# Autodesk Inventor assembly: Impresora 3D
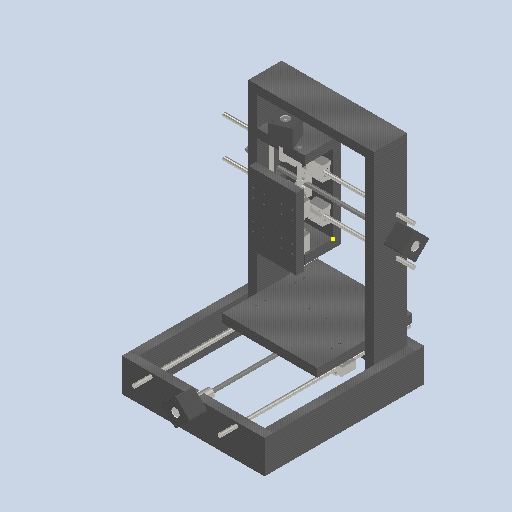
[picture p0: Inventor's stored thumbnail of the model, 512x512]
Saved by Autodesk Inventor 2022.2 (Build 262287000, 287)
## iProperties
Created: 2021-11-08
Part Number: Impresora 3D
Document SubType Name: Assembly
Designer: Samuel Gómez
Author: Samuel Gómez
## Documents named in this file (16)
- E:\Samuel Gómez\Documentos\ITM\Cuarto Semestre\Dibujo\Final\Original\Trabajo Final Impresora 3D\Impresora 3D.iam
- E:\Samuel Gómez\Documentos\ITM\Cuarto Semestre\Dibujo\Final\Original\Trabajo Final Impresora 3D\Placa1.ipt
- E:\Samuel Gómez\Documentos\ITM\Cuarto Semestre\Dibujo\Final\Original\Trabajo Final Impresora 3D\Placa2.ipt
- E:\Samuel Gómez\Documentos\ITM\Cuarto Semestre\Dibujo\Final\Original\Trabajo Final Impresora 3D\Placa1 Tracera.ipt
- E:\Samuel Gómez\Documentos\ITM\Cuarto Semestre\Dibujo\Final\Original\Trabajo Final Impresora 3D\Placa4 Torre.ipt
- E:\Samuel Gómez\Documentos\ITM\Cuarto Semestre\Dibujo\Final\Original\Trabajo Final Impresora 3D\Placa4 Torre Tracera.ipt
- E:\Samuel Gómez\Documentos\ITM\Cuarto Semestre\Dibujo\Final\Original\Trabajo Final Impresora 3D\Varrilla.ipt
- E:\Samuel Gómez\Documentos\ITM\Cuarto Semestre\Dibujo\Final\Original\Trabajo Final Impresora 3D\REFUERZO.ipt
- E:\Samuel Gómez\Documentos\ITM\Cuarto Semestre\Dibujo\Final\Original\Trabajo Final Impresora 3D\Balero lineal.ipt
- E:\Samuel Gómez\Documentos\ITM\Cuarto Semestre\Dibujo\Final\Original\Trabajo Final Impresora 3D\MOTOR.ipt
- E:\Samuel Gómez\Documentos\ITM\Cuarto Semestre\Dibujo\Final\Original\Trabajo Final Impresora 3D\ACOPLE FLEXIBLE.ipt
- E:\Samuel Gómez\Documentos\ITM\Cuarto Semestre\Dibujo\Final\Original\Trabajo Final Impresora 3D\Placa3 Cama.ipt
- E:\Samuel Gómez\Documentos\ITM\Cuarto Semestre\Dibujo\Final\Original\Trabajo Final Impresora 3D\CAMISA.ipt
- E:\Samuel Gómez\Documentos\ITM\Cuarto Semestre\Dibujo\Final\Original\Trabajo Final Impresora 3D\Extrusor.iam
- E:\Samuel Gómez\Documentos\ITM\Cuarto Semestre\Dibujo\Final\Original\Trabajo Final Impresora 3D\Placa5 Base Extrusor.ipt
- E:\Samuel Gómez\Documentos\ITM\Cuarto Semestre\Dibujo\Final\Original\Trabajo Final Impresora 3D\TORNILLO.ipt
## Components (36 placed, 15 different names)
1. Placa1:1 — Coincidencia:1, Nivelación:1, Nivelación:2, Nivelación:3, Nivelación:4, Coincidencia:2, Coincidencia:8, Coincidencia:9, Nivelación:9, Nivelación:10, Coincidencia:21, Coincidencia:22, Coincidencia:23
2. Placa2:1 — Coincidencia:1, Nivelación:1, Nivelación:2, Coincidencia:3, Coincidencia:4, Ángulo:3, Ángulo:4
3. Placa2:2 — Nivelación:3, Nivelación:4, Coincidencia:2, Nivelación:5, Nivelación:6, Coincidencia:6, Nivelación:8, Ángulo:1, Ángulo:2
4. Placa1 Tracera:1 — Coincidencia:3, Nivelación:5, Nivelación:6, Coincidencia:5, Nivelación:7, Coincidencia:7, Coincidencia:60
5. Placa4 Torre:1 — Coincidencia:4, Coincidencia:5, Nivelación:7, Nivelación:11, Nivelación:14, Coincidencia:24, Coincidencia:25, Coincidencia:26, Ángulo:11, Ángulo:12
6. Placa4 Torre Tracera:1 — Coincidencia:6, Coincidencia:7, Nivelación:8, Coincidencia:10, Coincidencia:11, Coincidencia:12, Nivelación:13, Ángulo:9, Ángulo:10, Coincidencia:61
7. Varrilla:1 — Coincidencia:8, Nivelación:10, Coincidencia:13, Coincidencia:14
8. Varrilla:2 — Coincidencia:9, Nivelación:9, Coincidencia:15, Coincidencia:16
9. Varrilla:3 — Coincidencia:10, Nivelación:11, Nivelación:12, Coincidencia:17, Coincidencia:19
10. Varrilla:4 — Coincidencia:11, Nivelación:12, Coincidencia:18, Coincidencia:20
11. Refuerzo:1 — Coincidencia:12, Nivelación:13, Nivelación:14, Ángulo:5, Ángulo:6, Ángulo:7, Ángulo:8
12. Balero lineal:1 — Coincidencia:13, Ángulo:1, Nivelación:16, Coincidencia:31
13. Balero lineal:2 — Coincidencia:14, Ángulo:2, Nivelación:15, Coincidencia:30, Coincidencia:60
14. Balero lineal:3 — Coincidencia:15, Ángulo:3, Nivelación:15
15. Balero lineal:4 — Coincidencia:16, Ángulo:4, Nivelación:16, Coincidencia:29
16. Balero lineal:5 — Coincidencia:18, Ángulo:6, Nivelación:17, Coincidencia:35, Coincidencia:36, Coincidencia:37
17. Balero lineal:6 — Coincidencia:17, Ángulo:5, Nivelación:17, Coincidencia:38
18. Balero lineal:7 — Coincidencia:20, Ángulo:7, Nivelación:18
19. Balero lineal:8 — Coincidencia:19, Ángulo:8, Nivelación:18, Coincidencia:39
20. Motor:1 — Coincidencia:21, Coincidencia:22, Coincidencia:23, Coincidencia:27, Nivelación:19
21. Motor:2 — Coincidencia:24, Coincidencia:25, Coincidencia:26, Coincidencia:28, Nivelación:20
22. Acople Flexible:1 — Coincidencia:27, Nivelación:19, Coincidencia:55, Coincidencia:56
23. Acople Flexible:2 — Coincidencia:28, Nivelación:20, Coincidencia:53, Coincidencia:54
24. Placa3 Cama:1 — Coincidencia:29, Coincidencia:30, Coincidencia:31, Coincidencia:32, Coincidencia:33, Coincidencia:34
25. Camisa:1 — Coincidencia:32, Coincidencia:33, Coincidencia:34
26. Extrusor:1 [sub-assembly] — Coincidencia:35, Coincidencia:36, Coincidencia:37, Coincidencia:38, Coincidencia:39, Coincidencia:40, Coincidencia:41, Coincidencia:42, Coincidencia:44, Coincidencia:45, Coincidencia:46, Coincidencia:47, Coincidencia:52, Coincidencia:57, Coincidencia:58, Coincidencia:59, Coincidencia:61
27. Motor:3 — Coincidencia:40, Coincidencia:41, Coincidencia:42, Coincidencia:43, Nivelación:21
28. Acople Flexible:3 — Coincidencia:43, Nivelación:21
29. Balero lineal:9 — Coincidencia:46, Ángulo:9, Nivelación:22
30. Balero lineal:10 — Coincidencia:45, Ángulo:12, Nivelación:23, Coincidencia:51, Coincidencia:52
31. Balero lineal:11 — Coincidencia:44, Ángulo:11, Nivelación:22, Coincidencia:48, Coincidencia:49, Coincidencia:50
32. Balero lineal:12 — Coincidencia:47, Ángulo:10, Nivelación:23
33. Placa5 Base Extrusor:1 — Coincidencia:48, Coincidencia:49, Coincidencia:50, Coincidencia:51
34. Tornillo:1 — Coincidencia:53, Coincidencia:54
35. Tornillo:2 — Coincidencia:55, Coincidencia:56
36. Camisa:2 — Coincidencia:57, Coincidencia:58, Coincidencia:59
## Relationships (96: Mate 61, Flush 23, Angle 12)
- Coincidencia:1 [Mate]: Placa1:1 ↔ Placa2:1
- Nivelación:1 [Flush]: Placa1:1 ↔ Placa2:1
- Nivelación:2 [Flush]: Placa1:1 ↔ Placa2:1
- Nivelación:3 [Flush]: Placa1:1 ↔ Placa2:2
- Nivelación:4 [Flush]: Placa1:1 ↔ Placa2:2
- Coincidencia:2 [Mate]: Placa1:1 ↔ Placa2:2
- Coincidencia:3 [Mate]: Placa2:1 ↔ Placa1 Tracera:1
- Nivelación:5 [Flush]: Placa2:2 ↔ Placa1 Tracera:1
- Nivelación:6 [Flush]: Placa2:2 ↔ Placa1 Tracera:1
- Coincidencia:4 [Mate]: Placa2:1 ↔ Placa4 Torre:1
- Coincidencia:5 [Mate]: Placa1 Tracera:1 ↔ Placa4 Torre:1
- Nivelación:7 [Flush]: Placa1 Tracera:1 ↔ Placa4 Torre:1
- Coincidencia:6 [Mate]: Placa2:2 ↔ Placa4 Torre Tracera:1
- Coincidencia:7 [Mate]: Placa1 Tracera:1 ↔ Placa4 Torre Tracera:1
- Nivelación:8 [Flush]: Placa2:2 ↔ Placa4 Torre Tracera:1
- Coincidencia:8 [Mate]: Placa1:1 ↔ Varrilla:1
- Coincidencia:9 [Mate]: Placa1:1 ↔ Varrilla:2
- Nivelación:9 [Flush] (-35 mm): Placa1:1 ↔ Varrilla:2
- Nivelación:10 [Flush] (-35 mm): Placa1:1 ↔ Varrilla:1
- Coincidencia:10 [Mate]: Placa4 Torre Tracera:1 ↔ Varrilla:3
- Nivelación:11 [Flush] (35 mm): Placa4 Torre:1 ↔ Varrilla:3
- Coincidencia:11 [Mate]: Placa4 Torre Tracera:1 ↔ Varrilla:4
- Nivelación:12 [Flush]: Varrilla:3 ↔ Varrilla:4
- Coincidencia:12 [Mate]: Placa4 Torre Tracera:1 ↔ Refuerzo:1
- Nivelación:13 [Flush]: Placa4 Torre Tracera:1 ↔ Refuerzo:1
- Nivelación:14 [Flush]: Placa4 Torre:1 ↔ Refuerzo:1
- Coincidencia:13 [Mate]: Varrilla:1 ↔ Balero lineal:1
- Coincidencia:14 [Mate]: Varrilla:1 ↔ Balero lineal:2
- Ángulo:1 [Angle] (0 deg): Placa2:2 ↔ Balero lineal:1
- Ángulo:2 [Angle] (0 deg): Placa2:2 ↔ Balero lineal:2
- Coincidencia:15 [Mate]: Varrilla:2 ↔ Balero lineal:3
- Coincidencia:16 [Mate]: Varrilla:2 ↔ Balero lineal:4
- Ángulo:3 [Angle] (0 deg): Placa2:1 ↔ Balero lineal:3
- Ángulo:4 [Angle] (0 deg): Placa2:1 ↔ Balero lineal:4
- Nivelación:15 [Flush]: Balero lineal:2 ↔ Balero lineal:3
- Nivelación:16 [Flush]: Balero lineal:1 ↔ Balero lineal:4
- Coincidencia:17 [Mate]: Varrilla:3 ↔ Balero lineal:6
- Coincidencia:18 [Mate]: Varrilla:4 ↔ Balero lineal:5
- Ángulo:5 [Angle] (0 deg): Refuerzo:1 ↔ Balero lineal:6
- Ángulo:6 [Angle] (0 deg): Refuerzo:1 ↔ Balero lineal:5
- Nivelación:17 [Flush]: Balero lineal:5 ↔ Balero lineal:6
- Coincidencia:19 [Mate]: Varrilla:3 ↔ Balero lineal:8
- Coincidencia:20 [Mate]: Varrilla:4 ↔ Balero lineal:7
- Ángulo:7 [Angle] (0 deg): Refuerzo:1 ↔ Balero lineal:7
- Ángulo:8 [Angle] (0 deg): Refuerzo:1 ↔ Balero lineal:8
- Nivelación:18 [Flush]: Balero lineal:7 ↔ Balero lineal:8
- Coincidencia:21 [Mate]: Placa1:1 ↔ Motor:1
- Coincidencia:22 [Mate]: Placa1:1 ↔ Motor:1
- Coincidencia:23 [Mate]: Placa1:1 ↔ Motor:1
- Coincidencia:24 [Mate]: Placa4 Torre:1 ↔ Motor:2
- Coincidencia:25 [Mate]: Placa4 Torre:1 ↔ Motor:2
- Coincidencia:26 [Mate]: Placa4 Torre:1 ↔ Motor:2
- Coincidencia:27 [Mate]: Motor:1 ↔ Acople Flexible:1
- Nivelación:19 [Flush]: Motor:1 ↔ Acople Flexible:1
- Coincidencia:28 [Mate]: Motor:2 ↔ Acople Flexible:2
- Nivelación:20 [Flush]: Motor:2 ↔ Acople Flexible:2
- Coincidencia:29 [Mate]: Balero lineal:4 ↔ Placa3 Cama:1
- Coincidencia:30 [Mate]: Balero lineal:2 ↔ Placa3 Cama:1
- Coincidencia:31 [Mate]: Balero lineal:1 ↔ Placa3 Cama:1
- Coincidencia:32 [Mate]: Placa3 Cama:1 ↔ Camisa:1
- Coincidencia:33 [Mate]: Placa3 Cama:1 ↔ Camisa:1
- Coincidencia:34 [Mate]: Placa3 Cama:1 ↔ Camisa:1
- Coincidencia:35 [Mate]: Balero lineal:5 ↔ Extrusor:1
- Coincidencia:36 [Mate]: Balero lineal:5 ↔ Extrusor:1
- Coincidencia:37 [Mate]: Balero lineal:5 ↔ Extrusor:1
- Coincidencia:38 [Mate]: Balero lineal:6 ↔ Extrusor:1
- Coincidencia:39 [Mate]: Balero lineal:8 ↔ Extrusor:1
- Coincidencia:40 [Mate]: Extrusor:1 ↔ Motor:3
- Coincidencia:41 [Mate]: Extrusor:1 ↔ Motor:3
- Coincidencia:42 [Mate]: Extrusor:1 ↔ Motor:3
- Coincidencia:43 [Mate]: Motor:3 ↔ Acople Flexible:3
- Nivelación:21 [Flush]: Motor:3 ↔ Acople Flexible:3
- Coincidencia:44 [Mate]: Extrusor:1 ↔ Balero lineal:11
- Coincidencia:45 [Mate]: Extrusor:1 ↔ Balero lineal:10
- Coincidencia:46 [Mate]: Extrusor:1 ↔ Balero lineal:9
- Coincidencia:47 [Mate]: Extrusor:1 ↔ Balero lineal:12
- Ángulo:9 [Angle] (0 deg): Placa4 Torre Tracera:1 ↔ Balero lineal:9
- Ángulo:10 [Angle] (0 deg): Placa4 Torre Tracera:1 ↔ Balero lineal:12
- Ángulo:11 [Angle] (0 deg): Placa4 Torre:1 ↔ Balero lineal:11
- Nivelación:22 [Flush]: Balero lineal:9 ↔ Balero lineal:11
- Ángulo:12 [Angle] (0 deg): Placa4 Torre:1 ↔ Balero lineal:10
- Nivelación:23 [Flush]: Balero lineal:10 ↔ Balero lineal:12
- Coincidencia:48 [Mate]: Balero lineal:11 ↔ Placa5 Base Extrusor:1
- Coincidencia:49 [Mate]: Balero lineal:11 ↔ Placa5 Base Extrusor:1
- Coincidencia:50 [Mate]: Balero lineal:11 ↔ Placa5 Base Extrusor:1
- Coincidencia:51 [Mate]: Balero lineal:10 ↔ Placa5 Base Extrusor:1
- Coincidencia:52 [Mate]: Extrusor:1 ↔ Balero lineal:10
- Coincidencia:53 [Mate]: Acople Flexible:2 ↔ Tornillo:1
- Coincidencia:54 [Mate]: Acople Flexible:2 ↔ Tornillo:1
- Coincidencia:55 [Mate]: Acople Flexible:1 ↔ Tornillo:2
- Coincidencia:56 [Mate]: Acople Flexible:1 ↔ Tornillo:2
- Coincidencia:57 [Mate]: Extrusor:1 ↔ Camisa:2
- Coincidencia:58 [Mate]: Extrusor:1 ↔ Camisa:2
- Coincidencia:59 [Mate]: Extrusor:1 ↔ Camisa:2
- Coincidencia:60 [Mate]: Placa1 Tracera:1 ↔ Balero lineal:2
- Coincidencia:61 [Mate]: Placa4 Torre Tracera:1 ↔ Extrusor:1
